# Autodesk Inventor assembly: 042
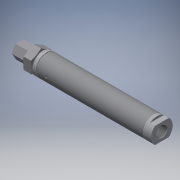
[picture p0: Inventor's stored thumbnail of the model, 180x180]
Saved by Autodesk Inventor 2018 (Build 220112000, 112)
## iProperties
Category: PARTsolutions
Company: BIMBA
Created: 2019-01-30
Part Number: 042
Catalog Web Link: www.cadenas.de
Description: Original Line Standard Air Cylinders-Standard Air Cylinders
Vendor: BIMBA
Document SubType Name: Assembly
Designer: psadmin
Manufacturer: BIMBA
PSOL_IDENT_0: {$CADENAS_DATA\23d-libs\bimba\bimba\bimba_imperial\bimba_full_line\original_line_cylinders\standard_
PSOL_IDENT_1: air_cylinders\standard_air_cylinder_asmtab.prj},314 {VTYP=3D},{STYP=ASSTAB},{NB=042},{LINA=042},{NN=
PSOL_IDENT_2: Original Line Standard Air Cylinders},{DATE=21.03.2018 14:31:21},{GEOMDATE=19.03.2018 11:39:15},{VER
PSOL_IDENT_3: SION=},{LINEID=50},{WBVAR=STROKE,ACTING,MNT,DER,NR,BM,CO,OO,VO,M,EE,EEL,K,Q,Y,G,T,HL,B,H,SER,SR,NT,W
PSOL_IDENT_4: ,STPT1,STPT2,STPT3,STPT4,MB,PB,PRC,TB,MN},{WBNUMERIC=STROKE,EEL}  {NB=042},{LINA=042},{KT=DUMMY},{PN=
PSOL_IDENT_5: 042},{PNC=042},{PNA=(NO ACCESSORIES)},{DASH=},{BORE1=0.75000000},{BORE=3/4\" (04)},{BOREPN=04},{STRO
PSOL_IDENT_6: KE=2.000},{STROKEALG=[0.011:50/0.001]},{STROKE1=2.000},{ACTING=},{ACTINGALG= '' , 'Single Acting (SA
PSOL_IDENT_7: )' , 'R' , 'Reverse Single Acting (SA)' , 'D' , 'Double Acting (SA)' },{ACTINGPN=},{MNT=},{MNTALG= ''
PSOL_IDENT_8: , 'Front Nose Mounting (SA)' , 'P' , 'Rear Pivot Mounting (SA)' , 'BF' , 'Front Block Mounting (SA)'
PSOL_IDENT_9: , 'BR' , 'Rear Block Mounting for Vertical Positioning (SA)' , 'BFT' , 'Front Block Trunnion Mounti
PSOL_IDENT_10: ng (SA)' , 'BRT' , 'Rear Block Trunnion Mounting (SA)' , 'A' , 'Double End Mounting with Brackets an
PSOL_IDENT_11: d Adjustable Stroke (SA)' , 'AP' , 'Rear Pivot Mounting with Adjustable Stroke (SA)' },{TYPE=},{MNTP
PSOL_IDENT_12: N=},{DER=},{DERALG= '' , 'N/A' },{NR=},{NRALG= '' , 'Round (Standard)' , 'NR' , 'Non-rotating - Hexa
PSOL_IDENT_13: gon Rod' },{NRPN=},{BM=},{BMALG= '' , 'Without Built-in Midget 3-Way Solenoid Operated Valve' , 'LS'
PSOL_IDENT_14: , 'With LS Series Solenoid Valve [LS]' },{BMPN=},{CO=},{COALG= '' , 'N/A' },{OO=},{OOALG= '', 'N/A'
PSOL_IDENT_15: },{OOPN=},{VO=Z},{VOALG= 'Z' , 'N/A' },{VOPN=},{OOVOPN=},{M=},{MALG= '', 'Without Magnet', 'M', 'Wi
PSOL_IDENT_16: th Magnet' },{EE=},{EEL=0.000},{EEMAX=48.0000},{EEALG= '', 'Without Extra Extension', 'EE', 'With Ex
PSOL_IDENT_17: tra Extension' },{EELALG=0},{EEPN=},{EEPN1=0.000},{K=},{KALG= '' , 'N/A' },{KPN=},{Q=},{QALG= '' , '
PSOL_IDENT_18: Standard Port' , 'Q' , 'Side Port' },{QPN=},{Y=},{YALG= '' , 'N/A' },{YPN=},{YCON=},{F=},{FALG= '', '
PSOL_IDENT_19: Non-Coated (Standard)', 'F', 'Molycoated' },{FPN=},{G=},{GPN=},{GPN99=},{T=},{TALG= '' , 'Standard -
PSOL_IDENT_20: 20° to 200°F (-29° to 95°C)' , 'N' , 'Low Temperature' , 'V' , 'High Temperature' },{NPN=},{VPN=},{H
PSOL_IDENT_21: L=},{HLALG= '' , 'N/A' },{B=},{BALG= '', 'W/out Bumpers' , 'B' , 'W/ Bumpers' },{BPN=},{H=},{HALG= ''
PSOL_IDENT_22: , 'W/ Standard Spring (Relaxed 3 lbs./Compressed 6 lbs.)', 'H', 'W/ Heavy Spring (Relaxed 4 lbs./Com
PSOL_IDENT_23: pressed 10 lbs.)' },{HPN=},{SER=},{SERALG= '' , 'N/A' },{SR=C},{SRALG= 'C' , 'Standard Blackened Car
PSOL_IDENT_24: bon Steel' , 'SR' , 'Stainless Steel [SR]' },{SRPN=},{SRCON=1},{NT=},{NTPN=},{W=},{WALG= '' , 'N/A'
PSOL_IDENT_25: },{WPN=},{E=},{EALG= '' , 'Standard Seals/Lube' , 'E' , 'Non-Lube Seals/Lube' },{EPN=},{ST=},{STALG=
PSOL_IDENT_26: '' , 'N/A' },{STPT1=},{STPT1ALG= '' , 'N/A' },{STPT2=},{STPT2ALG= '' , 'N/A' },{STPT3=},{STPT3ALG= ''
PSOL_IDENT_27: , 'N/A' },{STPT4=},{STPT4ALG= '' , 'N/A' },{STPN=},{MB=},{MBALG= '' , 'Without Mounting Bracket' , '
PSOL_IDENT_28: F,D-226' , 'D-226 (front)' },{MBPN=},{MBPNALL=D-226},{MBPNALLREAR=},{PB=},{PBALG= '' , 'N/A' },{PBPN=
PSOL_IDENT_29: },{PBPNALL=},{PRC=},{PRCALG= '' , 'W/out Pivot Rod Clevis' , 'F,D-166-3' , 'D-166-3 (front)' },{PRCP
PSOL_IDENT_30: N=},{PRCPNALL=D-166-3},{TB=},{TBALG= '' , 'N/A' },{TBPN=},{TBPNALL=},{MN=},{MNALG= '' , 'N/A' },{MNP
PSOL_IDENT_31: N=},{MNCONF=},{MNCONR=},{TLEN=3.9460},{FRAC=5.5700},{RGCON=},{RGDACCON=},{RHCON=},{RHCON1=},{RHCONON=
PSOL_IDENT_32: 1},{RHACCON=},{FNUTCON=1},{RNUTCON=0},{FNUTPN=D-98},{RNUTPN=},{FNUTTRANS=0.0000},{RNUTTRANS=0.0000},
PSOL_IDENT_33: {VHOLECON=2},{A1=0.8750},{A1N=0.8750},{A1P=1.5940},{A1B=1.5940},{A4=0.3130},{A4N=0.3130},{A4P=0.2525
PSOL_IDENT_34: },{A5=0.0300},{A1H=0.531},{A1NH=0.5310},{A1PH=1.5940},{A1BH=1.0940},{A1SH=1.2190},{A2H=0.2190},{A2NH=
PSOL_IDENT_35: 0.2190},{LENGTH=1.5000},{LENGTH1=1.5000},{LENGTH2=3.0300},{MUL=3.3800},{MUL11=3.3800},{MUL22=5.38},{
PSOL_IDENT_36: MUL33=3.3800},{MUL2=1.6900},{MUL211=1.6900},{MUL222=2.6900},{MUL233=1.6900},{SSS=4.0000},{RGLEN=0.59
PSOL_IDENT_37: 20},{RHLEN=0.3420},{SSS1=3.0000},{A13=1.3120},{DIF=0.0000},{G5=0.6250},{ON=0},{SSADD=0.0000},{BADD=0
PSOL_IDENT_38: .0000},{MADD=0.0000},{NVADD=0.0000},{TRACKL=3.6560},{TRACKCON=D-74168},{TRIMCON=0},{TRIMCON1=0},{PIN
PSOL_IDENT_39: CON=},{FSPACE=0.5786},{SPACE=0.0643},{TEXT=0.1125},{S1=1.0000},{D1=0.8050},{D1N=0.8050},{D1B=0.8625}
PSOL_IDENT_40: ,{D1P=0.8325},{FA=0.750},{RA=0.0000},{PPATH=standard_air_cylinder_asmtpl.prj},{MATALGHTML=<b>Standar
PSOL_IDENT_41: d Original Line:</b><dl><dt>Rod:</dt><dd>- Stainless Steel</dd><dd>&nbsp;&nbsp;(5/16 9/16 Bores)</dd
PSOL_IDENT_42: ><dd>- High Strength Carbon Steel</dd><dd>&nbsp;&nbsp;(3/4 3 Bore)</dd><dd>- Stainless Steel</dd><dd
PSOL_IDENT_43: >&nbsp;&nbsp;(X style DXP/DX/DXDE)</dd><dt>Bearings:</dt><dd>- Sintered Bronze</dd><dt>Body:</dt><dd
PSOL_IDENT_44: >- 304 Stainless Steel</dd><dt>End Caps:</dt><dd>- Aluminum</dd><dt>Seals:</dt><dd>- Buna N</dd></dl
PSOL_IDENT_45: >},{ASSCFGPRA=04},{MBPNA=},{MNPNA=},{PRCPNA=},{ASSOPTACC=STPT4},{A=4.88},{HADD=0.0000},{WFL=0.25},{Q
PSOL_IDENT_46: ADD=0.000},{QADD1=0.440},{TEST=2.0000},{MNTB=},{STDNUTF=1},{STDNUTR=0},{STRK2D=0},{X2D=2},{STROKESW=
PSOL_IDENT_47: 2.000},{EESW=0.000},{FCD=0},{BCD=0},{RCD=0},{CUSTADD=1.000},{FT=1/4-28 UNF-2A},{FT1=1/4-28 UNF-2A},{
PSOL_IDENT_48: FT2=5/8-18 UNF-2A},{PORT=1/8 NPT},{FT11=1/2-20 UNF-2A},{FT12=5/8-18 UNF-2A},{B1=}
NN: Original Line Standard Air Cylinders
NT: Standard Male Thread
NB: 042
NBSYN: $PNC.
LINA: 042
PN: 042
PNA: (NO ACCESSORIES)
BORE: 3/4" (04)
STROKE: 2
ACTING: Standard Single
MNT: Standard Front Nose
DER: N/A
NR: Standard Round
BM: Without Solenoid Operated Valve
CO: N/A
OO: N/A
VO: N/A
M: Without Magnet Piston
EE: Standard Rod Extension
EEL: 0
K: N/A
Q: Standard Axial Port
Y: N/A
G: Standard Grease Lube
T: Standard -20° to 200°F (-29° to 95°C)
HL: N/A
B: Without Bumpers
H: Standard (3 - 6 lbs.)
SER: N/A
SR: Standard Blackened Carbon Steel
W: N/A
STPT1: N/A
STPT2: N/A
STPT3: N/A
STPT4: N/A
MB: Without Mounting Bracket
PB: N/A
PRC: Without Piston Rod Clevis
TB: N/A
MN: N/A
A: 4.88
SUPPLIER: BIMBA
ARTICLENO: 042
BOMINFO: 042
CREATOR: CADENAS GmbH
Title: 042
Author: Cadenas PARTsolutions
Comments: Standard Air Cylinders
## Documents named in this file (8)
- C:\Users\maste\OneDrive\Documents\GitHub\2019CAD\Drivebase but Calvin is a mad man\AIS2018\042.iam
- C:\Users\maste\OneDrive\Documents\GitHub\2019CAD\Drivebase but Calvin is a mad man\AIS2018\042C0000000_0_dummy.ipt
- C:\Users\maste\OneDrive\Documents\GitHub\2019CAD\Drivebase but Calvin is a mad man\AIS2018\04000-0_rod_guide.ipt
- C:\Users\maste\OneDrive\Documents\GitHub\2019CAD\Drivebase but Calvin is a mad man\AIS2018\04-3_9462C.ipt
- C:\Users\maste\OneDrive\Documents\GitHub\2019CAD\Drivebase but Calvin is a mad man\AIS2018\040000_rear_head.ipt
- C:\Users\maste\OneDrive\Documents\GitHub\2019CAD\Drivebase but Calvin is a mad man\AIS2018\D-98.ipt
- C:\Users\maste\OneDrive\Documents\GitHub\2019CAD\Drivebase but Calvin is a mad man\AIS2018\C-0420000_rod.ipt
- C:\Users\maste\OneDrive\Documents\GitHub\2019CAD\Drivebase but Calvin is a mad man\Bevel Hex Shaft V2.ipt
## Components (7 placed, 7 different names)
1. 042C0000000_0_dummy:1
2. 04000-0_rod_guide:1 — Mate:1, Mate:4, Mate:6
3. 04-3_9462C:1
4. 040000_rear_head:1
5. D-98:1 — Mate:1, Mate:4
6. C-0420000_rod:1 — Mate:5
7. Bevel Hex Shaft V2:1 — Mate:5, Mate:6
## Relationships (4: Mate 4)
- Mate:1: 04000-0_rod_guide:1 ↔ D-98:1
- Mate:4 (1.5875 mm): 04000-0_rod_guide:1 ↔ D-98:1
- Mate:5: C-0420000_rod:1 ↔ Bevel Hex Shaft V2:1
- Mate:6: 04000-0_rod_guide:1 ↔ Bevel Hex Shaft V2:1
